# Autodesk Inventor assembly: 페그보드 조립
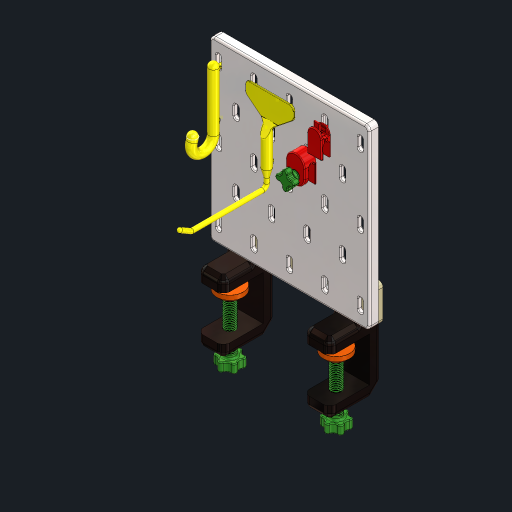
[picture p0: Inventor's stored thumbnail of the model, 512x512]
Saved by Autodesk Inventor 2024 (Build 280153000, 153)
## iProperties
Created: 2024-02-06
Part Number: 페그보드 조립
Document SubType Name: Assembly
Designer: KBU
Author: KBU
## Documents named in this file (11)
- D:\github\Modeling\IKEA 페그보드 시제품\SKÅDIS Pegboard assembly.iam
- D:\github\Modeling\IKEA 페그보드 시제품\Desk Clamp\SKÅDIS Pegboard Clamp.ipt
- D:\github\Modeling\IKEA 페그보드 시제품\SKÅDIS Pegboard\SKÅDIS Pegboard Front.ipt
- D:\github\Modeling\IKEA 페그보드 시제품\Desk Clamp\SKÅDIS Pegboard Clamp Addon.ipt
- D:\github\Modeling\IKEA 페그보드 시제품\Desk Clamp\SKÅDIS Pegboard Clamp Screw.ipt
- D:\github\Modeling\IKEA 페그보드 시제품\SKÅDIS Pegboard\SKÅDIS Pegboard Back.ipt
- D:\github\Modeling\IKEA 페그보드 시제품\Desk Clamp\SKÅDIS Pegboard Screw Cap.ipt
- D:\github\Modeling\IKEA 페그보드 시제품\Display Ring\상품걸이.ipt
- D:\github\Modeling\IKEA 페그보드 시제품\Display Ring\옷걸이ver2.ipt
- D:\github\Modeling\IKEA 페그보드 시제품\Clamp Vise\SKÅDIS Vise.iam
- D:\github\Modeling\IKEA 페그보드 시제품\Peg\SKÅDIS Pegboard Peg.iam
## Components (14 placed, 10 different names)
1. SKÅDIS Pegboard Front:1 — 메이트:7, 플러쉬:5, 플러쉬:6, 메이트:12, 메이트:13, 메이트:14, 메이트:15
2. SKÅDIS Pegboard Clamp Addon:1 — 메이트:3, 플러쉬:3, 메이트:4, 플러쉬:8, 메이트:9
3. SKÅDIS Pegboard Clamp:3 — 메이트:3, 플러쉬:3, 메이트:4, 원통형:2, 메이트:10
4. SKÅDIS Pegboard Clamp Addon:2 — 플러쉬:7, 메이트:8
5. SKÅDIS Pegboard Clamp:4 — 원통형:1, 메이트:11
6. SKÅDIS Pegboard Clamp Screw:1 — 원통형:1, 회전:2
7. SKÅDIS Pegboard Clamp Screw:2 — 원통형:2, 회전:1
8. SKÅDIS Pegboard Back:1 — 메이트:7, 플러쉬:5, 플러쉬:6, 플러쉬:7, 메이트:8, 플러쉬:8, 메이트:9
9. SKÅDIS Pegboard Screw Cap:1 — 회전:1, 메이트:10
10. SKÅDIS Pegboard Screw Cap:2 — 회전:2, 메이트:11
11. 상품걸이:1 — 메이트:13
12. 옷걸이ver2:1 — 메이트:12
13. SKÅDIS Vise:1 [sub-assembly] — 메이트:15
14. SKÅDIS Pegboard Peg:1 [sub-assembly] — 메이트:14
## Relationships (23: Mate 13, Flush 6, CylindricalJoint 2, RevoluteJoint 2)
- 메이트:3 [Mate] (0.125 mm): SKÅDIS Pegboard Clamp Addon:1 ↔ SKÅDIS Pegboard Clamp:3
- 플러쉬:3 [Flush]: SKÅDIS Pegboard Clamp Addon:1 ↔ SKÅDIS Pegboard Clamp:3
- 메이트:4 [Mate] (0.1 mm): SKÅDIS Pegboard Clamp Addon:1 ↔ SKÅDIS Pegboard Clamp:3
- [Mate] (0.125 mm): SKÅDIS Pegboard Clamp Addon:2 ↔ SKÅDIS Pegboard Clamp:4
- [Flush]: SKÅDIS Pegboard Clamp Addon:2 ↔ SKÅDIS Pegboard Clamp:4
- [Mate] (0.125 mm): SKÅDIS Pegboard Clamp Addon:2 ↔ SKÅDIS Pegboard Clamp:4
- 원통형:1 [CylindricalJoint]: SKÅDIS Pegboard Clamp:4 ↔ SKÅDIS Pegboard Clamp Screw:1
- 원통형:2 [CylindricalJoint]: SKÅDIS Pegboard Clamp:3 ↔ SKÅDIS Pegboard Clamp Screw:2
- 메이트:7 [Mate]: SKÅDIS Pegboard Front:1 ↔ SKÅDIS Pegboard Back:1
- 플러쉬:5 [Flush]: SKÅDIS Pegboard Front:1 ↔ SKÅDIS Pegboard Back:1
- 플러쉬:6 [Flush]: SKÅDIS Pegboard Front:1 ↔ SKÅDIS Pegboard Back:1
- 플러쉬:7 [Flush]: SKÅDIS Pegboard Clamp Addon:2 ↔ SKÅDIS Pegboard Back:1
- 메이트:8 [Mate]: SKÅDIS Pegboard Clamp Addon:2 ↔ SKÅDIS Pegboard Back:1
- 플러쉬:8 [Flush]: SKÅDIS Pegboard Clamp Addon:1 ↔ SKÅDIS Pegboard Back:1
- 메이트:9 [Mate]: SKÅDIS Pegboard Clamp Addon:1 ↔ SKÅDIS Pegboard Back:1
- 회전:1 [RevoluteJoint]: SKÅDIS Pegboard Clamp Screw:2 ↔ SKÅDIS Pegboard Screw Cap:1
- 회전:2 [RevoluteJoint]: SKÅDIS Pegboard Clamp Screw:1 ↔ SKÅDIS Pegboard Screw Cap:2
- 메이트:10 [Mate] (10 mm): SKÅDIS Pegboard Clamp:3 ↔ SKÅDIS Pegboard Screw Cap:1
- 메이트:11 [Mate] (10 mm): SKÅDIS Pegboard Clamp:4 ↔ SKÅDIS Pegboard Screw Cap:2
- 메이트:12 [Mate] (1 mm): SKÅDIS Pegboard Front:1 ↔ 옷걸이ver2:1
- 메이트:13 [Mate] (1 mm): SKÅDIS Pegboard Front:1 ↔ 상품걸이:1
- 메이트:14 [Mate]: SKÅDIS Pegboard Front:1 ↔ SKÅDIS Pegboard Peg:1
- 메이트:15 [Mate] (1 mm): SKÅDIS Pegboard Front:1 ↔ SKÅDIS Vise:1
## Named parameters: d27_d23 = 0.125 mm, d28_d24 = 0 mm, d29_d25 = 0.125 mm
